# Autodesk Inventor assembly: TEC Assembly
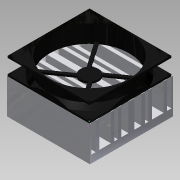
[picture p0: Inventor's stored thumbnail of the model, 180x180]
Saved by Autodesk Inventor 2015 (Build 190159000, 159)
## iProperties
Created: 2015-05-21
Part Number: TEC Assembly
Document SubType Name: Assembly
Designer: Joe Sheldon
Author: Joe Sheldon
## Documents named in this file (5)
- C:\Users\Joe Sheldon\Documents\PSU Stuff\PSU Clubs\Society of Physics Students\Cloud Chamber\Cloud Chamber CAD\TEC Unit\TEC Assembly.iam
- C:\Users\Joe Sheldon\Documents\PSU Stuff\PSU Clubs\Society of Physics Students\Cloud Chamber\Cloud Chamber CAD\TEC Unit\HeatSink.ipt
- C:\Users\Joe Sheldon\Documents\PSU Stuff\PSU Clubs\Society of Physics Students\Cloud Chamber\Cloud Chamber CAD\TEC Unit\fan_body.ipt
- C:\Users\Joe Sheldon\Documents\PSU Stuff\PSU Clubs\Society of Physics Students\Cloud Chamber\Cloud Chamber CAD\TEC Unit\peltier and mount.ipt
- C:\Users\Joe Sheldon\Documents\PSU Stuff\PSU Clubs\Society of Physics Students\Cloud Chamber\Cloud Chamber CAD\TEC Unit\peltier felt.ipt
## Components (4 placed, 4 different names)
1. HeatSink:1 — Rigid:1, Rigid:2
2. fan_body:1 — Rigid:1
3. peltier and mount:1 — Rigid:2, Rigid:3
4. peltier felt:1 — Rigid:3
## Relationships (3: WeldJoint 3)
- Rigid:1 [WeldJoint]: HeatSink:1 ↔ fan_body:1
- Rigid:2 [WeldJoint]: HeatSink:1 ↔ peltier and mount:1
- Rigid:3 [WeldJoint]: peltier and mount:1 ↔ peltier felt:1
